# Autodesk Inventor assembly: Flotador
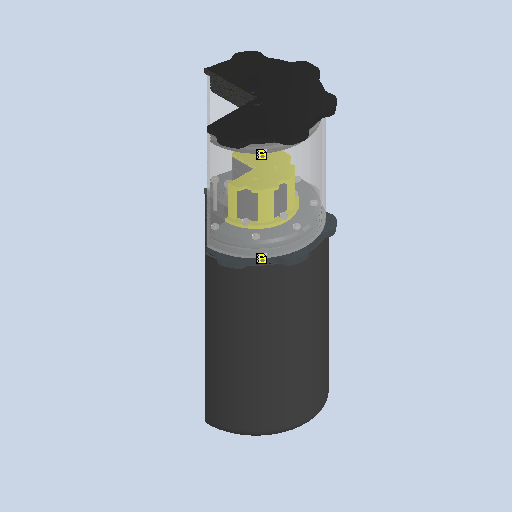
[picture p0: Inventor's stored thumbnail of the model, 512x512]
Saved by Autodesk Inventor 2025.3 (Build 293356030, 356C)
## iProperties
Created: 2025-10-11
Part Number: Flotador
Document SubType Name: Assembly
Designer: santa
Author: santa
## Documents named in this file (5)
- C:\Users\santa\OneDrive - Universidad de los Andes\Robocol\Flotador\V4\Flotador.iam
- C:\Users\santa\OneDrive - Universidad de los Andes\Robocol\Flotador\V4\Chasis.iam
- C:\Users\santa\OneDrive - Universidad de los Andes\Robocol\Flotador\V4\Expansor.iam
- C:\Users\santa\OneDrive\Documents\Inventor\Content Center Files\R2025\es-ES\ISO 4762(2)\ISO 4762 - M3 x 25ISO.ipt
- C:\Users\santa\OneDrive - Universidad de los Andes\Robocol\Flotador\V4\Capa\Capa.ipt
## Components (11 placed, 4 different names)
1. Chasis:1 [sub-assembly] — Nivelación:1, Nivelación:2, Nivelación:3, Rígido:1, Rígido:2, Rígido:3, Rígido:4, Rígido:5, Rígido:6, Rígido:7, Rígido:8, Coincidencia:3
2. Expansor:1 [sub-assembly] — Rígido:1, Coincidencia:2
3. Capa:1 — Coincidencia:2, Coincidencia:3
4. ISO 4762 M3 x 25:1 — Rígido:2
5. ISO 4762 M3 x 25:2 — Rígido:3
6. ISO 4762 M3 x 25:3 — Rígido:8
7. ISO 4762 M3 x 25:4 — Rígido:7
8. ISO 4762 M3 x 25:5 — Rígido:6
9. ISO 4762 M3 x 25:6 — Rígido:5
10. ISO 4762 M3 x 25:7 — Rígido:4
11. ISO 4762 M3 x 25:8
## Relationships (15: WeldJoint 8, Flush 3, Mate 3, Angle 1)
- Nivelación:1 [Flush]: Chasis:1
- Nivelación:2 [Flush]: Chasis:1
- Nivelación:3 [Flush]: Chasis:1
- Coincidencia:1 [Mate]
- Ángulo:1 [Angle] (30 deg)
- Rígido:1 [WeldJoint]: Chasis:1 ↔ Expansor:1
- Rígido:2 [WeldJoint]: Chasis:1 ↔ ISO 4762 M3 x 25:1
- Rígido:3 [WeldJoint]: Chasis:1 ↔ ISO 4762 M3 x 25:2
- Rígido:4 [WeldJoint]: Chasis:1 ↔ ISO 4762 M3 x 25:7
- Rígido:5 [WeldJoint]: Chasis:1 ↔ ISO 4762 M3 x 25:6
- Rígido:6 [WeldJoint]: Chasis:1 ↔ ISO 4762 M3 x 25:5
- Rígido:7 [WeldJoint]: Chasis:1 ↔ ISO 4762 M3 x 25:4
- Rígido:8 [WeldJoint]: Chasis:1 ↔ ISO 4762 M3 x 25:3
- Coincidencia:2 [Mate]: Expansor:1 ↔ Capa:1
- Coincidencia:3 [Mate]: Chasis:1 ↔ Capa:1
